# Autodesk Inventor assembly: Roller-ver1-1111-2019
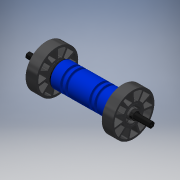
[picture p0: Inventor's stored thumbnail of the model, 180x180]
Saved by Autodesk Inventor 2018 (Build 220112000, 112)
## iProperties
Created: 2020-01-25
Part Number: Roller-ver1-1111-2019
Document SubType Name: Assembly
Designer: JMHal
Author: JMHal
## Documents named in this file (6)
- E:\GrabCAD\Power Hawks CAD\2020 Infinite Recharge\Storage\Assemblies\Roller-ver1-1111-2019.iam
- E:\GrabCAD\Power Hawks CAD\Resources\VEXpro Resources\Versa Motion\VersaHub(0.5inHex)-1111-2016.ipt
- E:\GrabCAD\Power Hawks CAD\2020 Infinite Recharge\Storage\Parts\Roller-ver3-1111-2019.ipt
- E:\GrabCAD\Power Hawks CAD\Resources\VEXpro Resources\Shafts\0.5inThunderHexShaft(8in(modified))-1111-2016.ipt
- E:\GrabCAD\Power Hawks CAD\Resources\VEXpro Resources\Wheels\4 inch\4IN-CompliantWheel-500Hex.iam
- E:\GrabCAD\Power Hawks CAD\Resources\VEXpro Resources\Spacers\0.25inAcetalSpacer(0.5inHex)-1111-2016.ipt
## Components (8 placed, 5 different names)
1. VersaHub(0.5inHex)-1111-2016:1 — Mate:12, Mate:13, Cylindrical:2, Mate:18
2. Roller-ver3-1111-2019:1 — Mate:10, Mate:11, Mate:12, Mate:13, Mate:16, Mate:19, Mate:22
3. VersaHub(0.5inHex)-1111-2016:2 — Mate:10, Mate:11, Mate:16, Mate:17, Mate:21
4. 0.5inThunderHexShaft(8in(modified))-1111-2016:1 — Cylindrical:1, Cylindrical:2, Flush:1
5. 0.25inAcetalSpacer(0.5inHex)-1111-2016:1 — Mate:17, Mate:23
6. 0.25inAcetalSpacer(0.5inHex)-1111-2016:2 — Cylindrical:1, Flush:1, Mate:20
7. 4IN-CompliantWheel-500Hex:1 [sub-assembly] — Mate:21, Mate:22, Mate:23
8. 4IN-CompliantWheel-500Hex:2 [sub-assembly] — Mate:18, Mate:19, Mate:20
## Relationships (15: Mate 12, CylindricalJoint 2, Flush 1)
- Mate:10: Roller-ver3-1111-2019:1 ↔ VersaHub(0.5inHex)-1111-2016:2
- Mate:11: Roller-ver3-1111-2019:1 ↔ VersaHub(0.5inHex)-1111-2016:2
- Mate:12: VersaHub(0.5inHex)-1111-2016:1 ↔ Roller-ver3-1111-2019:1
- Mate:13: VersaHub(0.5inHex)-1111-2016:1 ↔ Roller-ver3-1111-2019:1
- Cylindrical:1: 0.5inThunderHexShaft(8in(modified))-1111-2016:1 ↔ 0.25inAcetalSpacer(0.5inHex)-1111-2016:2
- Cylindrical:2: VersaHub(0.5inHex)-1111-2016:1 ↔ 0.5inThunderHexShaft(8in(modified))-1111-2016:1
- Mate:16: Roller-ver3-1111-2019:1 ↔ VersaHub(0.5inHex)-1111-2016:2
- Mate:17: VersaHub(0.5inHex)-1111-2016:2 ↔ 0.25inAcetalSpacer(0.5inHex)-1111-2016:1
- Flush:1 (38.1 mm): 0.5inThunderHexShaft(8in(modified))-1111-2016:1 ↔ 0.25inAcetalSpacer(0.5inHex)-1111-2016:2
- Mate:18: VersaHub(0.5inHex)-1111-2016:1 ↔ 4IN-CompliantWheel-500Hex:2
- Mate:19: Roller-ver3-1111-2019:1 ↔ 4IN-CompliantWheel-500Hex:2
- Mate:20: 0.25inAcetalSpacer(0.5inHex)-1111-2016:2 ↔ 4IN-CompliantWheel-500Hex:2
- Mate:21: VersaHub(0.5inHex)-1111-2016:2 ↔ 4IN-CompliantWheel-500Hex:1
- Mate:22: Roller-ver3-1111-2019:1 ↔ 4IN-CompliantWheel-500Hex:1
- Mate:23: 0.25inAcetalSpacer(0.5inHex)-1111-2016:1 ↔ 4IN-CompliantWheel-500Hex:1
